# Autodesk Inventor assembly: Drone_Launcher
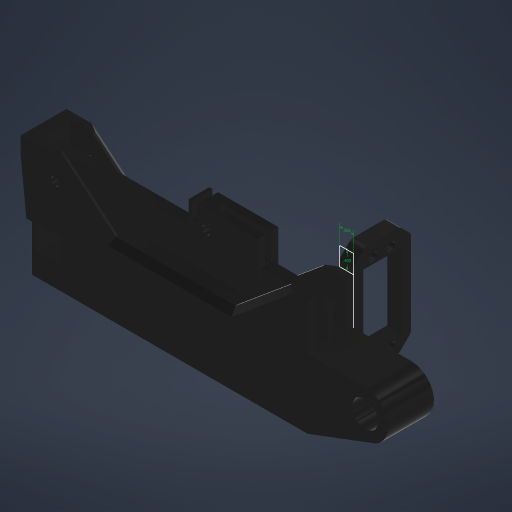
[picture p0: Inventor's stored thumbnail of the model, 512x512]
Saved by Autodesk Inventor 2023 (Build 270158000, 158)
## iProperties
Created: 2024-02-18
Part Number: Drone_Launcher
Document SubType Name: Assembly
Designer: kelle
Author: kelle
## Documents named in this file (4)
- C:\Users\kelle\OneDrive\Documents\Drone_Launcher.iam
- C:\Users\kelle\OneDrive\Documents\Drone_Launcher_Base.ipt
- C:\Users\kelle\OneDrive\Documents\Drone_Launcher_Carriage.ipt
- C:\Users\kelle\OneDrive\Documents\Drone_Launcher_Stopper.ipt
## Components (3 placed, 3 different names)
1. Drone_Launcher_Base:1 — Angle:1, Mate:1, Angle:2, Mate:2
2. Drone_Launcher_Carriage:1 — Angle:1, Mate:1
3. Drone_Launcher_Stopper:1 — Angle:2, Mate:2
## Relationships (4: Angle 2, Mate 2)
- Angle:1 (0 deg): Drone_Launcher_Base:1 ↔ Drone_Launcher_Carriage:1
- Mate:1: Drone_Launcher_Base:1 ↔ Drone_Launcher_Carriage:1
- Angle:2 (0 deg): Drone_Launcher_Base:1 ↔ Drone_Launcher_Stopper:1
- Mate:2: Drone_Launcher_Base:1 ↔ Drone_Launcher_Stopper:1
